# Autodesk Inventor assembly: OBG-Base Station v3
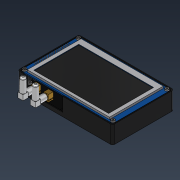
[picture p0: Inventor's stored thumbnail of the model, 180x180]
Saved by Autodesk Inventor 2022.1 (Build 261234020, 234B)
## iProperties
Part Number: OBG-Base Station v3
Material: Generisch
Document SubType Name: Assembly
Designer: rYan
Author: rYan
## Documents named in this file (4)
- D:\TIGERsGIT\Hardware\mechanik\2020\Inventor\Base Station\HBG-Base Station v3.iam
- D:\TIGERsGIT\Hardware\mechanik\2020\Inventor\Base Station\Gehaeuse BS v3.ipt
- D:\TIGERsGIT\Hardware\mechanik\2020\Inventor\Base Station\UBG-Electronics.iam
- D:\TIGERsGIT\Hardware\mechanik\2020\Inventor\Inhaltscenter\de-DE\DIN 7984\DIN 7984 - M3 x 5.ipt
## Components (9 placed, 3 different names)
1. Gehaeuse BS v3 Unten:1 — Fluchtend:1, Fluchtend:2, Fluchtend:3, Passend:1, Passend:2, Passend:3
2. UBG-Base Station v3:1 [sub-assembly] — Passend:1, Passend:2, Einfügen:1, Einfügen:2, Einfügen:3, Passend:3, Einfügen:4, Einfügen:5, Einfügen:6, Einfügen:7
3. DIN 7984 M3 x 5:1 — Einfügen:3
4. DIN 7984 M3 x 5:2 — Einfügen:2
5. DIN 7984 M3 x 5:3 — Einfügen:1
6. DIN 7984 M3 x 5:4 — Einfügen:4
7. DIN 7984 M3 x 5:5 — Einfügen:5
8. DIN 7984 M3 x 5:6 — Einfügen:6
9. DIN 7984 M3 x 5:7 — Einfügen:7
## Relationships (13: Insert 7, Flush 3, Mate 3)
- Fluchtend:1 [Flush]: Gehaeuse BS v3 Unten:1
- Fluchtend:2 [Flush]: Gehaeuse BS v3 Unten:1
- Fluchtend:3 [Flush]: Gehaeuse BS v3 Unten:1
- Passend:1 [Mate]: Gehaeuse BS v3 Unten:1 ↔ UBG-Base Station v3:1
- Passend:2 [Mate]: Gehaeuse BS v3 Unten:1 ↔ UBG-Base Station v3:1
- Einfügen:1 [Insert]: UBG-Base Station v3:1 ↔ DIN 7984 M3 x 5:3
- Einfügen:2 [Insert]: UBG-Base Station v3:1 ↔ DIN 7984 M3 x 5:2
- Einfügen:3 [Insert]: UBG-Base Station v3:1 ↔ DIN 7984 M3 x 5:1
- Passend:3 [Mate]: Gehaeuse BS v3 Unten:1 ↔ UBG-Base Station v3:1
- Einfügen:4 [Insert]: UBG-Base Station v3:1 ↔ DIN 7984 M3 x 5:4
- Einfügen:5 [Insert]: UBG-Base Station v3:1 ↔ DIN 7984 M3 x 5:5
- Einfügen:6 [Insert]: UBG-Base Station v3:1 ↔ DIN 7984 M3 x 5:6
- Einfügen:7 [Insert]: UBG-Base Station v3:1 ↔ DIN 7984 M3 x 5:7
